# Autodesk Inventor assembly: SCBRJ10-13
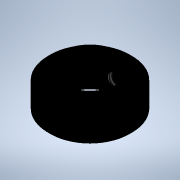
[picture p0: Inventor's stored thumbnail of the model, 180x180]
Saved by Autodesk Inventor 2021 (Build 250183000, 183)
## iProperties
Category: PARTsolutions
Company: MISUMI
Created: 2025-01-05
Part Number: SCBRJ10-13
Catalog Web Link: www.cadenas.de
Description: SCBRJ, PSCBRJ, SSCBRJ, SCSRAJ, SCSRAWJ, SCBSJ, PSCBSJ, SSCBSJ-Set Collars - For Bearing Fixing - (For Space Saving) - Set Screw Compact Type
Vendor: MISUMI
Document SubType Name: Assembly
Designer: psAdmin
Manufacturer: MISUMI
Mass: 0.947006 g
Surface Area: 9.73839 cm^2
Volume: 0.947006 cm^3
Density: 1 g/cm^3
Title: SCBRJ10-13
Author: Cadenas PARTsolutions
Comments: Set Collars - For Bearing Fixing - (For Space Saving) - Set Screw Compact Type
PSOL_IDENT_0: {$CADENAS_DATA/23d-libs/misumi/metric/03_set_collars/scbrj_asmtab.prj},245 {VTYP=3D},{STYP=ASSTAB},{
PSOL_IDENT_1: NB=SCBRJ10-13},{LINA=SCBRJ10-13},{NN=SCBRJ, PSCBRJ, SSCBRJ, SCSRAJ, SCSRAWJ, SCBSJ, PSCBSJ, SSCBSJ},
PSOL_IDENT_2: {DATE=02.11.2021 00:56:17},{GEOMDATE=19.10.2021 09:37:10},{VERSION=},{LINEID=60},{WBVAR=TS,MAT,ST,DS
PSOL_IDENT_3: S},{WBNUMERIC=DSS}  {NB=SCBRJ10-13},{LINA=SCBRJ10-13},{KT=DUMMY},{PN=SCBRJ10-13},{D=10},{TYPE=SCBRJ}
PSOL_IDENT_4: ,{TS=SN},{MAT=1045},{MATA='1045','1045 Carbon Steel','304','SUS304 Equivalent','2017','2017 Aluminum
PSOL_IDENT_5: Alloy'},{ST=Black Oxide},{AC=Set Screws 2 Pcs.},{DSS=13},{DS1=13,14,16},{AB=6800ZZ(19)},{B=7.5},{B1
PSOL_IDENT_6: 1=7.5},{B1=0},{B12=10},{D1=17},{M=M3x3},{THMD=3},{THDMIN=2.459},{BB=6},{ST0='Black Oxide','Black Oxi
PSOL_IDENT_7: de','Electroless Nickel Plating','Electroless Nickel Plating'},{C=0.5},{L=3},{TS1='SN','Short Nose','
PSOL_IDENT_8: LN','Long Nose'},{PPATH=scbrj/scbrj_templ.prj},{LTHREAD=3},{TIFF=1}
NB: SCBRJ10-13
NN: SCBRJ, PSCBRJ, SSCBRJ, SCSRAJ, SCSRAWJ, SCBSJ, PSCBSJ, SSCBSJ
NT: Set Collars - For Bearing Fixing - (For Space Saving) - Set Screw Compact Type
NBSYN: $PN.
LINA: SCBRJ10-13
CATALOG: Misumi
PN: SCBRJ10-13
D: 10
TS: Short Nose
MAT: 1045 Carbon Steel
ST: Black Oxide
AC: Set Screws 2 Pcs.
DSS: 13
AB: 6800ZZ(19)
B: 7.5
B1: 0
D1: 17
M: M3x3
BB: 6
SUPPLIER: MISUMI
ARTICLENO: SCBRJ10-13
BOMINFO: SCBRJ10-13
CREATOR: CADENAS GmbH
## Documents named in this file (3)
- e:\temp\worker_COMMON_641\temp\tmp_9988_14_2JYd6\format_0\SCBRJ10-13.iam
- e:\temp\worker_COMMON_641\temp\tmp_9988_14_2JYd6\format_0\SCBRJ10-13_b.ipt
- e:\temp\worker_COMMON_641\temp\tmp_9988_14_2JYd6\format_0\Hexagon socket set screw with flat point DIN 913 - M3x3.ipt
## Components (3 placed, 2 different names)
1. SCBRJ10-13_b:1 — body_set_v_Z@1 <-> IP1_Z@2, body_set_h_Z@1 <-> IP1_Z@3
2. Hexagon socket set screw with flat point DIN 913 - M3x3:1 — body_set_v_Z@1 <-> IP1_Z@2
3. Hexagon socket set screw with flat point DIN 913 - M3x3:2 — body_set_h_Z@1 <-> IP1_Z@3
## Relationships (2: Mate 2)
- body_set_v_Z@1 <-> IP1_Z@2 [Mate]: SCBRJ10-13_b:1 ↔ Hexagon socket set screw with flat point DIN 913 - M3x3:1
- body_set_h_Z@1 <-> IP1_Z@3 [Mate]: SCBRJ10-13_b:1 ↔ Hexagon socket set screw with flat point DIN 913 - M3x3:2
